# Autodesk Inventor assembly: interface
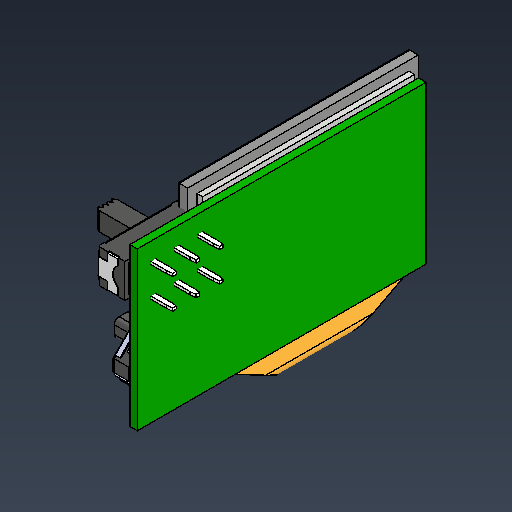
[picture p0: Inventor's stored thumbnail of the model, 512x512]
Saved by Autodesk Inventor 2026.2 (Build 302298010, 298A)
## iProperties
Created: 2026-03-25
Part Number: interface
Document SubType Name: Assembly
Designer: szymo
Author: szymo
## Documents named in this file (5)
- D:\tech\robotyka\robots\evangelion-turbo\inventor-project\interface.iam
- D:\tech\robotyka\robots\evangelion-turbo\inventor-project\0.96 oled\0.96 oled\0.96 oled.ipt
- D:\tech\robotyka\robots\evangelion-turbo\inventor-project\microswitch_EG1271A\microswitch_EG1271A\microswitch_EG1271A.ipt
- D:\tech\robotyka\robots\evangelion-turbo\inventor-project\THMU 13 (SMD JOYSTICK)\THMU 13 (SMD JOYSTICK)\THMU 13 (SMD JOYSTICK).ipt
- D:\tech\robotyka\robots\evangelion-turbo\inventor-project\interface-pcb.ipt
## Components (4 placed, 4 different names)
1. interface-pcb:1 — Mate:1, Mate:2, Flush:2, Mate:3
2. THMU 13 (SMD JOYSTICK):1
3. microswitch_EG1271A:1
4. 0.96 oled:1
## Relationships (4: Mate 3, Flush 1)
- Mate:1: interface-pcb:1
- Mate:2: interface-pcb:1
- Flush:2: interface-pcb:1
- Mate:3: interface-pcb:1
